# Autodesk Inventor assembly: EX_ONE
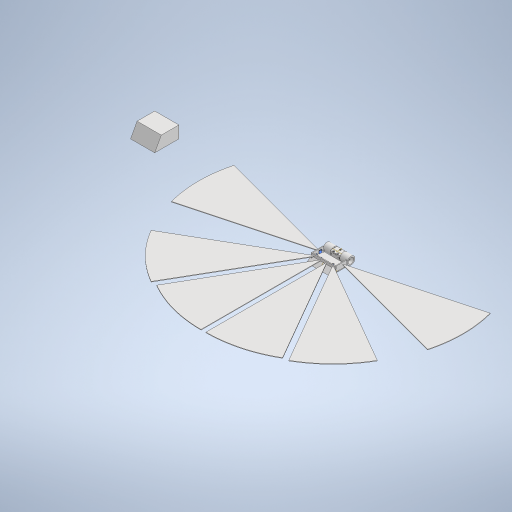
[picture p0: Inventor's stored thumbnail of the model, 512x512]
Saved by Autodesk Inventor 2023 (Build 270158000, 158)
## iProperties
Created: 2025-01-11
Part Number: EX_ONE
Document SubType Name: Assembly
Designer: kamil
Author: kamil
## Documents named in this file (12)
- C:\Users\kamil\Documents\PROJECTS - repos\EX_ONE_minisumo\mechanics\inventor_parts\EX_ONE.iam
- C:\Users\kamil\Documents\PROJECTS - repos\EX_ONE_minisumo\mechanics\inventor_parts\faulhaber_motor.ipt
- C:\Users\kamil\Documents\PROJECTS - repos\EX_ONE_minisumo\mechanics\inventor_parts\motors_mount.ipt
- C:\Users\kamil\Documents\PROJECTS - repos\EX_ONE_minisumo\mechanics\inventor_parts\kolo_tetsowe.ipt
- C:\Users\kamil\Documents\PROJECTS - repos\EX_ONE_minisumo\mechanics\inventor_parts\podstawa.ipt
- C:\Users\kamil\Documents\PROJECTS - repos\EX_ONE_minisumo\mechanics\inventor_parts\nóź.ipt
- C:\Users\kamil\Documents\PROJECTS - repos\EX_ONE_minisumo\mechanics\inventor_parts\TOF_VL53L0X (1).ipt
- C:\Users\kamil\Documents\PROJECTS - repos\EX_ONE_minisumo\mechanics\inventor_parts\pcb_pre.ipt
- C:\Users\kamil\Documents\PROJECTS - repos\EX_ONE_minisumo\mechanics\inventor_parts\minisunmo_testowe.ipt
- C:\Users\kamil\Documents\PROJECTS - repos\EX_ONE_minisumo\mechanics\inventor_parts\ściana.ipt
- C:\Users\kamil\Documents\PROJECTS - repos\EX_ONE_minisumo\mechanics\inventor_parts\ściana_MIR.ipt
- C:\Users\kamil\Documents\PROJECTS - repos\EX_ONE_minisumo\mechanics\inventor_parts\przod.ipt
## Components (18 placed, 11 different names)
1. faulhaber_motor:1 — Kątowe:1, Zestawiające:1, Zestawiające:2, Zestawiające:4, Równoległe:2
2. faulhaber_motor:2 — Kątowe:1, Zestawiające:1, Zestawiające:2, Równoległe:1, Zestawiające:3
3. motors_mount:1 — Równoległe:1, Zestawiające:3, Zestawiające:7, Równoległe:4, Zestawiające:9, Zestawiające:13
4. kolo_tetsowe:1 — Zestawiające:4, Równoległe:2, Równoległe:3
5. podstawa:1 — Zestawiające:7, Równoległe:3, Równoległe:4, Równoległe:5, Równoległe:6, Równoległe:7, Równoległe:8, Zestawiające:10, Równoległe:9, Kątowe:2, Zestawiające:12, Równoległe:16, Równoległe:17, Równoległe:19, Równoległe:20, Zestawiające:15
6. nóź:1 — Równoległe:5, Równoległe:6
7. kolo_tetsowe:2 — Równoległe:7, Zestawiające:9
8. pcb_pre:1 — Równoległe:8, Zestawiające:10, Równoległe:9, Zestawiające:11, Kątowe:6, Równoległe:18
9. TOF_VL53L0X (1):1 — Zestawiające:11, Równoległe:10, Równoległe:11, Równoległe:12, Równoległe:15, Równoległe:18, Zestawiające:17
10. TOF_VL53L0X (1):2 — Równoległe:11, Równoległe:15, Zestawiające:16
11. TOF_VL53L0X (1):3 — Równoległe:10, Równoległe:14, Kątowe:2, Kątowe:5, Zestawiające:13, Zestawiające:14
12. TOF_VL53L0X (1):4 — Równoległe:12, Równoległe:13, Kątowe:4, Kątowe:6, Zestawiające:14
13. TOF_VL53L0X (1):5 — Równoległe:13, Kątowe:4
14. TOF_VL53L0X (1):6 — Równoległe:14, Kątowe:5
15. minisunmo_testowe:1
16. ściana:1 — Zestawiające:12, Równoległe:16, Równoległe:17, Zestawiające:17, Zestawiające:18, Równoległe:21, Zestawiające:19
17. ściana_MIR:1 — Równoległe:19, Równoległe:20, Zestawiające:15, Zestawiające:16
18. przod:1 — Zestawiające:18, Równoległe:21, Zestawiające:19
## Relationships (42: Flush 21, Mate 16, Angle 5)
- Kątowe:1 [Angle] (180 deg): faulhaber_motor:1 ↔ faulhaber_motor:2
- Zestawiające:1 [Mate]: faulhaber_motor:1 ↔ faulhaber_motor:2
- Zestawiające:2 [Mate] (6.6 mm): faulhaber_motor:1 ↔ faulhaber_motor:2
- Równoległe:1 [Flush]: faulhaber_motor:2 ↔ motors_mount:1
- Zestawiające:3 [Mate]: faulhaber_motor:2 ↔ motors_mount:1
- Zestawiające:4 [Mate]: faulhaber_motor:1 ↔ kolo_tetsowe:1
- Równoległe:2 [Flush] (15 mm): faulhaber_motor:1 ↔ kolo_tetsowe:1
- Zestawiające:7 [Mate]: motors_mount:1 ↔ podstawa:1
- Równoległe:3 [Flush]: kolo_tetsowe:1 ↔ podstawa:1
- Równoległe:4 [Flush] (1 mm): motors_mount:1 ↔ podstawa:1
- Równoległe:5 [Flush]: podstawa:1 ↔ nóź:1
- Równoległe:6 [Flush] (3.25 mm): podstawa:1 ↔ nóź:1
- Równoległe:7 [Flush]: podstawa:1 ↔ kolo_tetsowe:2
- Zestawiające:9 [Mate]: motors_mount:1 ↔ kolo_tetsowe:2
- Równoległe:8 [Flush] (-8 mm): podstawa:1 ↔ pcb_pre:1
- Zestawiające:10 [Mate] (3 mm): podstawa:1 ↔ pcb_pre:1
- Równoległe:9 [Flush] (-2 mm): podstawa:1 ↔ pcb_pre:1
- Zestawiające:11 [Mate]: pcb_pre:1 ↔ TOF_VL53L0X (1):1
- Równoległe:10 [Flush]: TOF_VL53L0X (1):1 ↔ TOF_VL53L0X (1):3
- Równoległe:11 [Flush]: TOF_VL53L0X (1):1 ↔ TOF_VL53L0X (1):2
- Równoległe:12 [Flush]: TOF_VL53L0X (1):1 ↔ TOF_VL53L0X (1):4
- Równoległe:13 [Flush]: TOF_VL53L0X (1):4 ↔ TOF_VL53L0X (1):5
- Równoległe:14 [Flush]: TOF_VL53L0X (1):3 ↔ TOF_VL53L0X (1):6
- Równoległe:15 [Flush]: TOF_VL53L0X (1):1 ↔ TOF_VL53L0X (1):2
- Kątowe:2 [Angle] (15 deg): podstawa:1 ↔ TOF_VL53L0X (1):3
- Kątowe:4 [Angle] (-30 deg): TOF_VL53L0X (1):4 ↔ TOF_VL53L0X (1):5
- Kątowe:5 [Angle] (30 deg): TOF_VL53L0X (1):3 ↔ TOF_VL53L0X (1):6
- Zestawiające:12 [Mate]: podstawa:1 ↔ ściana:1
- Równoległe:16 [Flush]: podstawa:1 ↔ ściana:1
- Równoległe:17 [Flush]: podstawa:1 ↔ ściana:1
- Kątowe:6 [Angle] (0 deg): pcb_pre:1 ↔ TOF_VL53L0X (1):4
- Zestawiające:13 [Mate] (10 mm): motors_mount:1 ↔ TOF_VL53L0X (1):3
- Zestawiające:14 [Mate] (20 mm): TOF_VL53L0X (1):3 ↔ TOF_VL53L0X (1):4
- Równoległe:18 [Flush] (2 mm): pcb_pre:1 ↔ TOF_VL53L0X (1):1
- Równoległe:19 [Flush]: podstawa:1 ↔ ściana_MIR:1
- Równoległe:20 [Flush]: podstawa:1 ↔ ściana_MIR:1
- Zestawiające:15 [Mate]: podstawa:1 ↔ ściana_MIR:1
- Zestawiające:16 [Mate]: TOF_VL53L0X (1):2 ↔ ściana_MIR:1
- Zestawiające:17 [Mate]: TOF_VL53L0X (1):1 ↔ ściana:1
- Zestawiające:18 [Mate]: ściana:1 ↔ przod:1
- Równoległe:21 [Flush]: ściana:1 ↔ przod:1
- Zestawiające:19 [Mate]: ściana:1 ↔ przod:1
